# Autodesk Inventor assembly: LiftPrototypeMKI
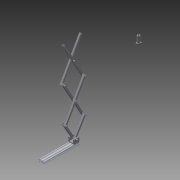
[picture p0: Inventor's stored thumbnail of the model, 180x180]
Saved by Autodesk Inventor 2013 (Build 170138000, 138)
## iProperties
Created: 2013-10-02
Part Number: LiftPrototypeMKI
Document SubType Name: Assembly
Designer: cobrooks
Author: cobrooks
## Documents named in this file (10)
- C:\Users\cobrooks\Documents\Robotics\2013-14\CAD\Lift\LiftPrototype\LiftPrototypeMKI.iam
- \\lmss\STUDENTS\Robotics\CAD Files\5x5mm Box Aluminum.ipt
- \\lmss\STUDENTS\Robotics\CAD Files\COTS Parts\Fasteners\14-20 Washer - Flat.ipt
- \\lmss\STUDENTS\Robotics\CAD Files\COTS Parts\Fasteners\8-32 BHCS x1500.ipt
- \\lmss\STUDENTS\Robotics\CAD Files\COTS Parts\Fasteners\8-32 locknut.ipt
- \\lmss\STUDENTS\Robotics\CAD Files\ShortBox.ipt
- \\lmss\STUDENTS\Robotics\CAD Files\COTS Parts\Bosch Extrusion\Bosch 20x40.ipt
- \\lmss\STUDENTS\Robotics\CAD Files\4150 Robot 2013-2014\LiftPrototype\LiftBase2.ipt
- \\lmss\STUDENTS\Robotics\CAD Files\COTS Parts\Fasteners\8-32 BHCS x2000.ipt
- \\lmss\STUDENTS\Robotics\CAD Files\4150 Robot 2013-2014\LiftPrototype\ScrewShaft.ipt
## Components (32 placed, 9 different names)
1. 14-20 Washer - Flat:1 — Insert:2, Insert:3
2. 5x5mm Box Aluminum:1 — Insert:1, Insert:2, Insert:12, Insert:15, Insert:20, Insert:23
3. 5x5mm Box Aluminum:2 — Insert:3, Insert:4, Insert:11, Insert:16, Insert:18, Insert:22
4. 8-32 BHCS x1500:1 — Insert:1, Mate:5
5. 8-32 locknut:1 — Insert:4
6. 5x5mm Box Aluminum:3 — Insert:5, Insert:6, Insert:9, Insert:13
7. 5x5mm Box Aluminum:4 — Insert:7, Insert:8, Insert:10, Insert:14
8. 8-32 BHCS x1500:2 — Insert:5, Mate:6
9. 8-32 locknut:2 — Insert:8
10. 14-20 Washer - Flat:3 — Insert:6, Insert:7
11. 14-20 Washer - Flat:4 — Insert:17, Insert:18
12. 8-32 BHCS x1500:3 — Insert:21
13. 8-32 locknut:3 — Insert:22
14. 14-20 Washer - Flat:5 — Insert:9, Insert:12
15. 14-20 Washer - Flat:6 — Insert:10, Insert:11
16. 8-32 BHCS x1500:4 — Insert:13
17. 8-32 BHCS x1500:5 — Insert:14
18. 8-32 locknut:4 — Insert:15
19. 8-32 locknut:5 — Insert:16
20. ShortBox:1 — Insert:17, Insert:21, Insert:25, Insert:27
21. ShortBox:2 — Insert:19, Insert:24, Insert:26, Insert:28
22. 14-20 Washer - Flat:7 — Insert:19, Insert:20
23. 8-32 locknut:6 — Insert:24
24. 8-32 BHCS x1500:6 — Insert:23
25. 14-20 Washer - Flat:8 — Insert:25, Insert:26
26. Bosch 20x40:1 — Mate:1, Mate:2, Flush:1, Flush:2
27. LiftBase2:2 — Insert:29, Insert:30, Insert:31, Mate:2, Flush:1, Flush:2
28. 14-20 Washer - Flat:10 — Insert:28
29. 14-20 Washer - Flat:11 — Insert:27, Insert:29
30. 8-32 BHCS x2000:1 — Insert:30, Mate:3, Mate:4
31. 8-32 locknut:8 — Insert:31
32. ScrewShaft:1
## Relationships (39: Insert 31, Mate 6, Flush 2)
- Insert:1: 5x5mm Box Aluminum:1 ↔ 8-32 BHCS x1500:1
- Insert:2: 14-20 Washer - Flat:1 ↔ 5x5mm Box Aluminum:1
- Insert:3: 14-20 Washer - Flat:1 ↔ 5x5mm Box Aluminum:2
- Insert:4: 5x5mm Box Aluminum:2 ↔ 8-32 locknut:1
- Insert:5: 5x5mm Box Aluminum:3 ↔ 8-32 BHCS x1500:2
- Insert:6: 5x5mm Box Aluminum:3 ↔ 14-20 Washer - Flat:3
- Insert:7: 5x5mm Box Aluminum:4 ↔ 14-20 Washer - Flat:3
- Insert:8: 5x5mm Box Aluminum:4 ↔ 8-32 locknut:2
- Insert:9: 5x5mm Box Aluminum:3 ↔ 14-20 Washer - Flat:5
- Insert:10: 5x5mm Box Aluminum:4 ↔ 14-20 Washer - Flat:6
- Insert:11: 5x5mm Box Aluminum:2 ↔ 14-20 Washer - Flat:6
- Insert:12: 5x5mm Box Aluminum:1 ↔ 14-20 Washer - Flat:5
- Insert:13: 5x5mm Box Aluminum:3 ↔ 8-32 BHCS x1500:4
- Insert:14: 5x5mm Box Aluminum:4 ↔ 8-32 BHCS x1500:5
- Insert:15: 5x5mm Box Aluminum:1 ↔ 8-32 locknut:4
- Insert:16: 5x5mm Box Aluminum:2 ↔ 8-32 locknut:5
- Insert:17: 14-20 Washer - Flat:4 ↔ ShortBox:1
- Insert:18: 5x5mm Box Aluminum:2 ↔ 14-20 Washer - Flat:4
- Insert:19: ShortBox:2 ↔ 14-20 Washer - Flat:7
- Insert:20: 5x5mm Box Aluminum:1 ↔ 14-20 Washer - Flat:7
- Insert:21: 8-32 BHCS x1500:3 ↔ ShortBox:1
- Insert:22: 5x5mm Box Aluminum:2 ↔ 8-32 locknut:3
- Insert:23: 5x5mm Box Aluminum:1 ↔ 8-32 BHCS x1500:6
- Insert:24: ShortBox:2 ↔ 8-32 locknut:6
- Mate:1: Bosch 20x40:1
- Insert:25: ShortBox:1 ↔ 14-20 Washer - Flat:8
- Insert:26: ShortBox:2 ↔ 14-20 Washer - Flat:8
- Insert:27: ShortBox:1 ↔ 14-20 Washer - Flat:11
- Insert:28: ShortBox:2 ↔ 14-20 Washer - Flat:10
- Insert:29: LiftBase2:2 ↔ 14-20 Washer - Flat:11
- Insert:30: LiftBase2:2 ↔ 8-32 BHCS x2000:1
- Insert:31: LiftBase2:2 ↔ 8-32 locknut:8
- Mate:2: Bosch 20x40:1 ↔ LiftBase2:2
- Flush:1: Bosch 20x40:1 ↔ LiftBase2:2
- Flush:2: Bosch 20x40:1 ↔ LiftBase2:2
- Mate:3: 8-32 BHCS x2000:1
- Mate:4: 8-32 BHCS x2000:1
- Mate:5: 8-32 BHCS x1500:1
- Mate:6: 8-32 BHCS x1500:2
